# Autodesk Inventor assembly: Top joint housing back
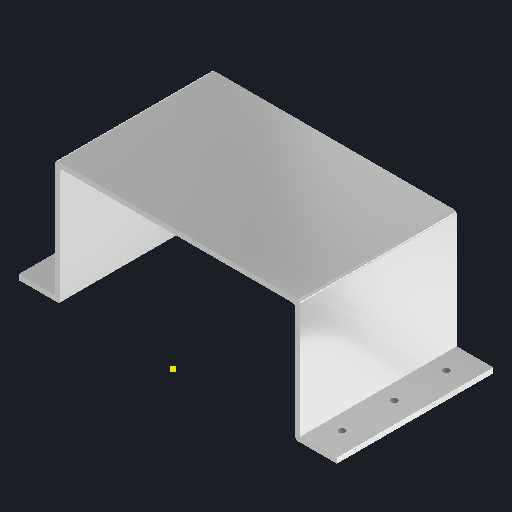
[picture p0: Inventor's stored thumbnail of the model, 512x512]
Saved by Autodesk Inventor 2026.3 (Build 303398000, 398)
## iProperties
Created: 2026-07-28
Part Number: Top joint housing back
Document SubType Name: Assembly
Designer: matot
Author: matot
## Documents named in this file (3)
- C:\Users\matot\OneDrive - Stellenbosch University\2026\MechatronicsProject478\Building the joint\Joint Assembly\Top joint housing back.iam
- C:\Users\matot\OneDrive - Stellenbosch University\2026\MechatronicsProject478\Building the joint\Joint Assembly\Top joint housing back.ipt
- C:\Users\matot\OneDrive - Stellenbosch University\2026\MechatronicsProject478\Building the joint\Joint Assembly\Joint housing cover.ipt
## Components (2 placed, 2 different names)
1. Top joint housing back:1 — Mate:1, Flush:1, Flush:2, Mate:2
2. Joint housing cover:1 — Mate:1, Flush:1, Flush:2, Mate:2
## Relationships (4: Mate 2, Flush 2)
- Mate:1: Top joint housing back:1 ↔ Joint housing cover:1
- Flush:1: Top joint housing back:1 ↔ Joint housing cover:1
- Flush:2: Top joint housing back:1 ↔ Joint housing cover:1
- Mate:2: Top joint housing back:1 ↔ Joint housing cover:1
